# Autodesk Inventor assembly: RIGHT ARM
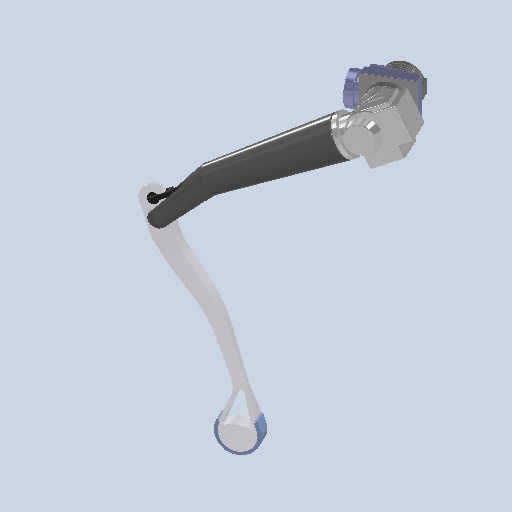
[picture p0: Inventor's stored thumbnail of the model, 512x512]
Saved by Autodesk Inventor 2023 (Build 270158000, 158)
## iProperties
Created: 2022-11-08
Part Number: RIGHT ARM
Document SubType Name: Assembly
Designer: willy
Author: willy
## Documents named in this file (7)
- C:\Users\willy\Documents\SPOT\RIGHT ARM.iam
- C:\Users\willy\Documents\SPOT\motor1_v2.ipt
- C:\Users\willy\Documents\SPOT\motor2.ipt
- C:\Users\willy\Documents\SPOT\motor3+fan(rignt).ipt
- C:\Users\willy\Documents\SPOT\spot_arm_v2.ipt
- C:\Users\willy\Documents\SPOT\spot_foot.ipt
- C:\Users\willy\Documents\SPOT\joint_v2.ipt
## Components (6 placed, 6 different names)
1. motor1_v2:1 — 메이트:1, 메이트:2, 삽입:1, 삽입:2
2. motor2:1 — 메이트:1, 메이트:2, 삽입:1
3. motor3+fan(rignt):1 — 삽입:2, 메이트:3, 삽입:3
4. spot_arm_v2:1 — 메이트:3, 삽입:3, 삽입:4, 메이트:4
5. spot_foot:1 — 삽입:4, 삽입:5
6. joint_v2:1 — 삽입:5, 메이트:4
## Relationships (9: Insert 5, Mate 4)
- 메이트:1 [Mate]: motor1_v2:1 ↔ motor2:1
- 메이트:2 [Mate]: motor1_v2:1 ↔ motor2:1
- 삽입:1 [Insert]: motor1_v2:1 ↔ motor2:1
- 삽입:2 [Insert]: motor1_v2:1 ↔ motor3+fan(rignt):1
- 메이트:3 [Mate]: motor3+fan(rignt):1 ↔ spot_arm_v2:1
- 삽입:3 [Insert]: motor3+fan(rignt):1 ↔ spot_arm_v2:1
- 삽입:4 [Insert]: spot_arm_v2:1 ↔ spot_foot:1
- 삽입:5 [Insert]: spot_foot:1 ↔ joint_v2:1
- 메이트:4 [Mate]: spot_arm_v2:1 ↔ joint_v2:1
